# Autodesk Inventor assembly: Assy
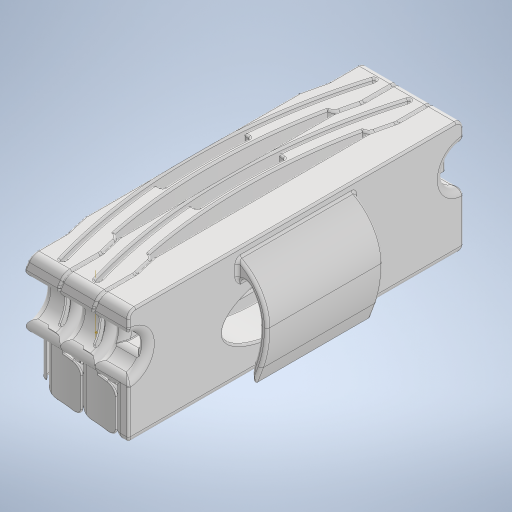
[picture p0: Inventor's stored thumbnail of the model, 512x512]
Saved by Autodesk Inventor 2024 (Build 280153000, 153)
## iProperties
Created: 2024-12-25
Part Number: Assy
Document SubType Name: Assembly
Designer: rrenkit
Author: rrenkit
## Documents named in this file (4)
- C:\Users\rrenkit\OneDrive\Portfolio\2024 - ClipOn Sunglasses Holder\CAD\V2\Assy.iam
- C:\Users\rrenkit\OneDrive\Portfolio\2024 - ClipOn Sunglasses Holder\CAD\V2\housing.ipt
- C:\Users\rrenkit\OneDrive\Portfolio\2024 - ClipOn Sunglasses Holder\CAD\V2\clip.ipt
- C:\Users\rrenkit\Documents\CAD\Clip-On Sunglasses Holder\V2\bracket.ipt
## Components (4 placed, 3 different names)
1. housing:1 — Mate:1, Flush:1, Mate:2
2. housing:2 — Mate:1, Flush:1, Mate:2, Mate:3, Mate:4, Mate:5
3. clip:1 — Mate:3, Mate:4, Mate:5, Angle:1, Mate:15, Mate:16
4. bracket:1 — Mate:15, Mate:16
## Relationships (10: Mate 8, Flush 1, Angle 1)
- Mate:1: housing:1 ↔ housing:2
- Flush:1: housing:1 ↔ housing:2
- Mate:2: housing:1 ↔ housing:2
- Mate:3: housing:2 ↔ clip:1
- Mate:4: housing:2 ↔ clip:1
- Mate:5: housing:2 ↔ clip:1
- Angle:1 (0 deg): clip:1
- Mate:14
- Mate:15: clip:1 ↔ bracket:1
- Mate:16: clip:1 ↔ bracket:1
